# Autodesk Inventor assembly: 000.100 - Манипулятор
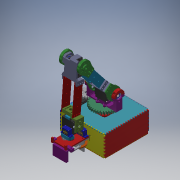
[picture p0: Inventor's stored thumbnail of the model, 180x180]
Saved by Autodesk Inventor 2019 (Build 230136000, 136)
## iProperties
Created: 2020-02-23
Part Number: 000.100 - Манипулятор
Material: Типовые
Document SubType Name: Assembly
Designer: Петров Иван
Author: Петров Иван
## Documents named in this file (11)
- E:\IVAN\Ivan_desktop\Kvantorium\Competitions\INOP_2020\hardware\5-DOF\000.100 - Манипулятор.iam
- E:\IVAN\Ivan_desktop\Kvantorium\Competitions\INOP_2020\hardware\5-DOF\000.200 - Короб электроники.iam
- E:\IVAN\Ivan_desktop\Kvantorium\Competitions\INOP_2020\hardware\5-DOF\000.300 - Опора поворотная.iam
- E:\IVAN\Ivan_desktop\Kvantorium\Competitions\INOP_2020\hardware\5-DOF\components\Star Horn MG995.ipt
- E:\IVAN\Ivan_desktop\Kvantorium\Competitions\INOP_2020\hardware\5-DOF\000.100 - Манипулятор\Мастер проектирования\Цилиндрическое зубчатое зацепление1.iam
- E:\IVAN\Ivan_desktop\Kvantorium\Competitions\INOP_2020\hardware\5-DOF\000.303 - Шестерня привода.ipt
- E:\IVAN\Ivan_desktop\Kvantorium\Competitions\INOP_2020\hardware\5-DOF\000.400 - Первое звено.iam
- E:\IVAN\Ivan_desktop\Kvantorium\Competitions\INOP_2020\hardware\5-DOF\000.500 - Второе звено.iam
- E:\IVAN\Ivan_desktop\Kvantorium\Competitions\INOP_2020\hardware\5-DOF\000.600 - Третье звездо.iam
- E:\IVAN\Ivan_desktop\Kvantorium\Competitions\INOP_2020\hardware\5-DOF\000.700 - Крепеж захвата.iam
- E:\IVAN\Ivan_desktop\Kvantorium\Competitions\INOP_2020\hardware\5-DOF\000.800 - Захват.iam
## Components (10 placed, 10 different names)
1. 000.200 - Короб электроники:1 [sub-assembly] — Совмещение:1, Совмещение:2, Совмещение:3, Совмещение:4, Совмещение:5, Ограничитель горизонтального поворота, Ограничитель первого сочленения, Угол инструмента, Совмещение:29
2. 000.300 - Опора поворотная:1 [sub-assembly] — Совмещение:1, Совмещение:2, Совмещение:3, Совмещение:12, Совмещение:13, Совмещение:14, Совмещение:25, Совмещение:26, Совмещение:27
3. Star Horn MG995:1 — Совмещение:4, Совмещение:5, Совмещение:24, Совмещение:28, Совмещение:30
4. Цилиндрическое зубчатое зацепление:1 [sub-assembly] — Совмещение:24, Совмещение:25, Совмещение:26, Совмещение:27
5. 000.303 - Шестерня привода:1 — Совмещение:28, Совмещение:29, Совмещение:30
6. 000.400 - Первое звено:1 [sub-assembly] — Совмещение:12, Совмещение:13, Совмещение:14, Совмещение:15, Совмещение:16, Совмещение:17, Ограничитель горизонтального поворота, Ограничитель первого сочленения, Ограничитель второго сочленения
7. 000.500 - Второе звено:1 [sub-assembly] — Совмещение:15, Совмещение:16, Совмещение:17, Ограничитель второго сочленения, Совмещение:18, Совмещение:19, Совмещение:20
8. 000.600 - Третье звездо:1 [sub-assembly] — Совмещение:18, Совмещение:19, Совмещение:20, Совмещение:21, Совмещение:22, Совмещение:23, Угол:5
9. 000.700 - Крепеж захвата:1 [sub-assembly] — Совмещение:21, Совмещение:22, Совмещение:23, Угол инструмента, Совмещение:31, Совмещение:32, Совмещение:33
10. 000.800 - Захват:1 [sub-assembly] — Совмещение:31, Совмещение:32, Совмещение:33, Угол:5
## Relationships (32: Mate 27, Angle 5)
- Совмещение:1 [Mate]: 000.200 - Короб электроники:1 ↔ 000.300 - Опора поворотная:1
- Совмещение:2 [Mate]: 000.200 - Короб электроники:1 ↔ 000.300 - Опора поворотная:1
- Совмещение:3 [Mate]: 000.200 - Короб электроники:1 ↔ 000.300 - Опора поворотная:1
- Совмещение:4 [Mate]: 000.200 - Короб электроники:1 ↔ Star Horn MG995:1
- Совмещение:5 [Mate]: 000.200 - Короб электроники:1 ↔ Star Horn MG995:1
- Совмещение:12 [Mate]: 000.300 - Опора поворотная:1 ↔ 000.400 - Первое звено:1
- Совмещение:13 [Mate]: 000.300 - Опора поворотная:1 ↔ 000.400 - Первое звено:1
- Совмещение:14 [Mate]: 000.300 - Опора поворотная:1 ↔ 000.400 - Первое звено:1
- Совмещение:15 [Mate]: 000.400 - Первое звено:1 ↔ 000.500 - Второе звено:1
- Совмещение:16 [Mate]: 000.400 - Первое звено:1 ↔ 000.500 - Второе звено:1
- Совмещение:17 [Mate]: 000.400 - Первое звено:1 ↔ 000.500 - Второе звено:1
- Ограничитель горизонтального поворота [Angle] (0 deg): 000.200 - Короб электроники:1 ↔ 000.400 - Первое звено:1
- Ограничитель первого сочленения [Angle] (0 deg): 000.200 - Короб электроники:1 ↔ 000.400 - Первое звено:1
- Ограничитель второго сочленения [Angle] (-90 deg): 000.400 - Первое звено:1 ↔ 000.500 - Второе звено:1
- Совмещение:18 [Mate]: 000.500 - Второе звено:1 ↔ 000.600 - Третье звездо:1
- Совмещение:19 [Mate]: 000.500 - Второе звено:1 ↔ 000.600 - Третье звездо:1
- Совмещение:20 [Mate]: 000.500 - Второе звено:1 ↔ 000.600 - Третье звездо:1
- Совмещение:21 [Mate]: 000.600 - Третье звездо:1 ↔ 000.700 - Крепеж захвата:1
- Совмещение:22 [Mate]: 000.600 - Третье звездо:1 ↔ 000.700 - Крепеж захвата:1
- Совмещение:23 [Mate]: 000.600 - Третье звездо:1 ↔ 000.700 - Крепеж захвата:1
- Угол инструмента [Angle] (-90 deg): 000.200 - Короб электроники:1 ↔ 000.700 - Крепеж захвата:1
- Совмещение:24 [Mate]: Star Horn MG995:1 ↔ Цилиндрическое зубчатое зацепление:1
- Совмещение:25 [Mate]: 000.300 - Опора поворотная:1 ↔ Цилиндрическое зубчатое зацепление:1
- Совмещение:26 [Mate]: 000.300 - Опора поворотная:1 ↔ Цилиндрическое зубчатое зацепление:1
- Совмещение:27 [Mate]: 000.300 - Опора поворотная:1 ↔ Цилиндрическое зубчатое зацепление:1
- Совмещение:28 [Mate]: Star Horn MG995:1 ↔ 000.303 - Шестерня привода:1
- Совмещение:29 [Mate]: 000.200 - Короб электроники:1 ↔ 000.303 - Шестерня привода:1
- Совмещение:30 [Mate]: Star Horn MG995:1 ↔ 000.303 - Шестерня привода:1
- Совмещение:31 [Mate]: 000.700 - Крепеж захвата:1 ↔ 000.800 - Захват:1
- Совмещение:32 [Mate]: 000.700 - Крепеж захвата:1 ↔ 000.800 - Захват:1
- Совмещение:33 [Mate]: 000.700 - Крепеж захвата:1 ↔ 000.800 - Захват:1
- Угол:5 [Angle] (0 deg): 000.600 - Третье звездо:1 ↔ 000.800 - Захват:1
